# Autodesk Inventor assembly: GANTRY & FRAME ASSY
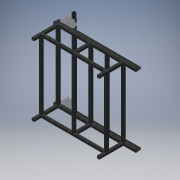
[picture p0: Inventor's stored thumbnail of the model, 180x180]
Saved by Autodesk Inventor 2018 (Build 220112000, 112)
## iProperties
Created: 2018-10-15
Part Number: GANTRY & FRAME ASSY
Material: Genérico
Document SubType Name: Assembly
Designer: Toshiba
Author: Toshiba
## Documents named in this file (3)
- C:\U\Semestre Primavera 2018\Diseño de sistemas mecánicos\CNC\DiseñoCNC\Gantry\GANTRY & FRAME ASSY.iam
- C:\U\Semestre Primavera 2018\Diseño de sistemas mecánicos\CNC\DiseñoCNC\Gantry\STEEL FRAME & RAILS ASSY.iam
- C:\U\Semestre Primavera 2018\Diseño de sistemas mecánicos\CNC\DiseñoCNC\Gantry\GANTRY.iam
## Components (2 placed, 2 different names)
1. STEEL FRAME & RAILS ASSY:1 [sub-assembly] — Tangente:1, Tangente:2, Tangente:3, Tangente:4, Tangente:5, Tangente:6
2. GANTRY:1 [sub-assembly] — Tangente:1, Tangente:2, Tangente:3, Tangente:4, Tangente:5, Tangente:6
## Relationships (6: Tangent 6)
- Tangente:1: STEEL FRAME & RAILS ASSY:1 ↔ GANTRY:1
- Tangente:2: STEEL FRAME & RAILS ASSY:1 ↔ GANTRY:1
- Tangente:3: STEEL FRAME & RAILS ASSY:1 ↔ GANTRY:1
- Tangente:4: STEEL FRAME & RAILS ASSY:1 ↔ GANTRY:1
- Tangente:5: STEEL FRAME & RAILS ASSY:1 ↔ GANTRY:1
- Tangente:6: STEEL FRAME & RAILS ASSY:1 ↔ GANTRY:1
